# Autodesk Inventor assembly: FinalRev1
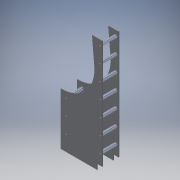
[picture p0: Inventor's stored thumbnail of the model, 180x180]
Saved by Autodesk Inventor 2016 (Build 200138000, 138)
## iProperties
Created: 2017-01-22
Part Number: FinalRev1
Document SubType Name: Assembly
Designer: madsenn
Author: madsenn
## Documents named in this file (3)
- C:\Users\madsenn\Documents\GitHub\Robot2017\Assemblies\FinalRev1.iam
- C:\Users\madsenn\Documents\GitHub\Robot2017\LauncherSidePlate.ipt
- C:\Users\madsenn\Documents\GitHub\Robot2017\Parts\3InchChurro.ipt
## Components (12 placed, 2 different names)
1. LauncherSidePlate:1 — Mate:3, Mate:4, Mate:5, Mate:6, Mate:7, Mate:8, Mate:9, Mate:10, Mate:11, Mate:12, Mate:13, Mate:14, Mate:15, Mate:16, Mate:17, Mate:18, Mate:19, Mate:20, Mate:21, Mate:22
2. LauncherSidePlate:2 — Mate:1, Mate:2, Mate:23, Mate:24, Mate:25, Mate:26, Mate:27, Mate:28, Mate:29, Mate:30, Mate:31
3. 3InchChurro:1 — Mate:5, Mate:6, Mate:23
4. 3InchChurro:2 — Mate:7, Mate:8, Mate:24
5. 3InchChurro:3 — Mate:21, Mate:22, Mate:29
6. 3InchChurro:4 — Mate:9, Mate:10, Mate:25
7. 3InchChurro:5 — Mate:11, Mate:12, Mate:26
8. 3InchChurro:6 — Mate:15, Mate:16, Mate:28
9. 3InchChurro:7 — Mate:13, Mate:14, Mate:27
10. 3InchChurro:8 — Mate:17, Mate:18, Mate:31
11. 3InchChurro:9 — Mate:19, Mate:20, Mate:30
12. 3InchChurro:10 — Mate:1, Mate:2, Mate:3, Mate:4
## Relationships (31: Mate 31)
- Mate:1: LauncherSidePlate:2 ↔ 3InchChurro:10
- Mate:2: LauncherSidePlate:2 ↔ 3InchChurro:10
- Mate:3: LauncherSidePlate:1 ↔ 3InchChurro:10
- Mate:4: LauncherSidePlate:1 ↔ 3InchChurro:10
- Mate:5: LauncherSidePlate:1 ↔ 3InchChurro:1
- Mate:6: LauncherSidePlate:1 ↔ 3InchChurro:1
- Mate:7: LauncherSidePlate:1 ↔ 3InchChurro:2
- Mate:8: LauncherSidePlate:1 ↔ 3InchChurro:2
- Mate:9: LauncherSidePlate:1 ↔ 3InchChurro:4
- Mate:10: LauncherSidePlate:1 ↔ 3InchChurro:4
- Mate:11: LauncherSidePlate:1 ↔ 3InchChurro:5
- Mate:12: LauncherSidePlate:1 ↔ 3InchChurro:5
- Mate:13: LauncherSidePlate:1 ↔ 3InchChurro:7
- Mate:14: LauncherSidePlate:1 ↔ 3InchChurro:7
- Mate:15: LauncherSidePlate:1 ↔ 3InchChurro:6
- Mate:16: LauncherSidePlate:1 ↔ 3InchChurro:6
- Mate:17: LauncherSidePlate:1 ↔ 3InchChurro:8
- Mate:18: LauncherSidePlate:1 ↔ 3InchChurro:8
- Mate:19: LauncherSidePlate:1 ↔ 3InchChurro:9
- Mate:20: LauncherSidePlate:1 ↔ 3InchChurro:9
- Mate:21: LauncherSidePlate:1 ↔ 3InchChurro:3
- Mate:22: LauncherSidePlate:1 ↔ 3InchChurro:3
- Mate:23: LauncherSidePlate:2 ↔ 3InchChurro:1
- Mate:24: LauncherSidePlate:2 ↔ 3InchChurro:2
- Mate:25: LauncherSidePlate:2 ↔ 3InchChurro:4
- Mate:26: LauncherSidePlate:2 ↔ 3InchChurro:5
- Mate:27: LauncherSidePlate:2 ↔ 3InchChurro:7
- Mate:28: LauncherSidePlate:2 ↔ 3InchChurro:6
- Mate:29: LauncherSidePlate:2 ↔ 3InchChurro:3
- Mate:30: LauncherSidePlate:2 ↔ 3InchChurro:9
- Mate:31: LauncherSidePlate:2 ↔ 3InchChurro:8
